# Autodesk Inventor assembly: assy_straight
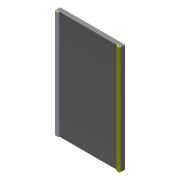
[picture p0: Inventor's stored thumbnail of the model, 180x180]
Saved by Autodesk Inventor 2018 (Build 220112000, 112)
## iProperties
Created: 2017-11-13
Part Number: assy_straight
Document SubType Name: Assembly
Designer: Platform
Author: Platform
## Documents named in this file (3)
- C:\Users\Platform\Desktop\autorace_track\track_model\autorace_rbizchallenge2017\assembled\assy_straight.iam
- C:\Users\Platform\Desktop\autorace_track\track_model\autorace_rbizchallenge2017\parts\ipt\upper_plate_straight v1.ipt
- C:\Users\Platform\Desktop\autorace_track\track_model\autorace_rbizchallenge2017\parts\ipt\straight_line.ipt
## Components (3 placed, 2 different names)
1. upper_plate_straight v1:1
2. straight_line:1
3. straight_line:2
## Relationships (4: Mate 4)
- [Mate]: upper_plate_straight v1:1 ↔ straight_line:1
- [Mate]: upper_plate_straight v1:1 ↔ straight_line:1
- [Mate]: upper_plate_straight v1:1 ↔ straight_line:2
- [Mate]: upper_plate_straight v1:1 ↔ straight_line:2
